# Autodesk Inventor assembly: Assembly1
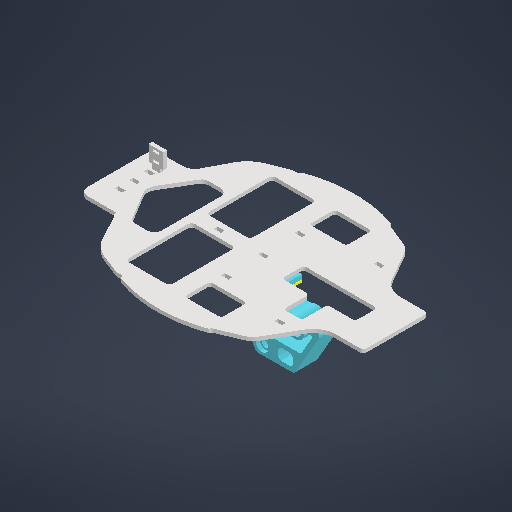
[picture p0: Inventor's stored thumbnail of the model, 512x512]
Saved by Autodesk Inventor 2025.3 (Build 293356000, 356)
## iProperties
Created: 2025-11-12
Part Number: Assembly1
Document SubType Name: Assembly
Designer: sophi
Author: sophi
## Documents named in this file (4)
- C:\Users\sophi\OneDrive - Universidad de los andes\Documentos\1 Universidad\5 Semestre\Proyecto\Huron-Hudson\Pelton Engine\V12\Assembly1.iam
- C:\Users\sophi\OneDrive - Universidad de los andes\Documentos\1 Universidad\5 Semestre\Proyecto\Base proyecto intermedio.ipt
- C:\Users\sophi\OneDrive - Universidad de los andes\Documentos\1 Universidad\5 Semestre\Proyecto\Huron-Hudson\Pelton Engine\V12\base.ipt
- C:\Users\sophi\OneDrive - Universidad de los andes\Documentos\1 Universidad\5 Semestre\Proyecto\Huron-Hudson\Pelton Engine\V12\fizer.ipt
## Components (3 placed, 3 different names)
1. Base proyecto intermedio:1 — Flush:1, Flush:2, Flush:3, Mate:1
2. base:1 — Mate:1, Mate:3, Mate:4
3. fizer:1 — Mate:3, Mate:4
## Relationships (6: Flush 3, Mate 3)
- Flush:1: Base proyecto intermedio:1
- Flush:2: Base proyecto intermedio:1
- Flush:3: Base proyecto intermedio:1
- Mate:1: Base proyecto intermedio:1 ↔ base:1
- Mate:3: base:1 ↔ fizer:1
- Mate:4: base:1 ↔ fizer:1
